# Autodesk Inventor assembly: pc053_33
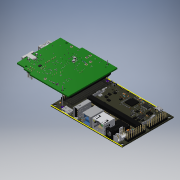
[picture p0: Inventor's stored thumbnail of the model, 180x180]
Saved by Autodesk Inventor 2017 (Build 210142000, 142)
## iProperties
Created: 2016-10-24
Part Number: pc053_33
Document SubType Name: Assembly
Designer: phpgb
Author: phpgb
## Documents named in this file (4)
- P:\cad\designs\uob-hep-pc053a\trunk\design_files\worklib\pc053a_toplevel\physical\3DModel\pc053_33.iam
- P:\cad\designs\uob-hep-pc053a\trunk\design_files\worklib\pc053a_toplevel\physical\3DModel\pc053a_toplevel_33.iam
- P:\cad\steps_files\FMCblankFrontPanel10.ipt
- O:\Documents\Inventor\Enclustra\Mars_PM3.iam
## Components (3 placed, 3 different names)
1. pc053a_toplevel_33:1 [sub-assembly] — Mate:1, Mate:2, Angle:1, Mate:3, Mate:4
2. FMCblankFrontPanel10:1 — Mate:1, Mate:2, Angle:1
3. Mars_PM3:1 [sub-assembly] — Mate:3, Mate:4
## Relationships (5: Mate 4, Angle 1)
- Mate:1: pc053a_toplevel_33:1 ↔ FMCblankFrontPanel10:1
- Mate:2: pc053a_toplevel_33:1 ↔ FMCblankFrontPanel10:1
- Angle:1 (0 deg): pc053a_toplevel_33:1 ↔ FMCblankFrontPanel10:1
- Mate:3: pc053a_toplevel_33:1 ↔ Mars_PM3:1
- Mate:4: pc053a_toplevel_33:1 ↔ Mars_PM3:1
